# Autodesk Inventor assembly: Spool Holder V2.1
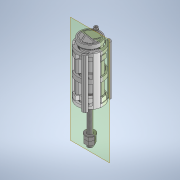
[picture p0: Inventor's stored thumbnail of the model, 180x180]
Saved by Autodesk Inventor 2020.3 (Build 243373010, 373A)
## iProperties
Created: 2021-07-05
Part Number: Spool Holder V2.1
Document SubType Name: Assembly
Designer: Parker
Author: Parker
## Documents named in this file (57)
- D:\Designs\MK3PRO P1\ACCESSORIES\Spool Holder V2\Spool Holder V2.1.iam
- D:\Designs\MK3PRO P1\ACCESSORIES\Spool Holder V2\M8 All Thread.ipt
- D:\Designs\MK3PRO P1\ACCESSORIES\Spool Holder V2\M8 Nut 6.ipt
- D:\Designs\MK3PRO P1\ACCESSORIES\Spool Holder V2\608RS Bearing.ipt
- D:\Designs\MK3PRO P1\ACCESSORIES\Spool Holder V2\M8 Washer.ipt
- D:\Designs\MK3PRO P1\ACCESSORIES\Spool Holder V2\M8 Nut 1.ipt
- D:\Designs\MK3PRO P1\ACCESSORIES\Spool Holder V2\M8 Washer 2.ipt
- D:\Designs\MK3PRO P1\ACCESSORIES\Spool Holder V2\M8 Nut 2.ipt
- D:\Designs\MK3PRO P1\ACCESSORIES\Spool Holder V2\M8 Nut 3.ipt
- D:\Designs\MK3PRO P1\ACCESSORIES\Spool Holder V2\M8 Washer 3.ipt
- D:\Designs\MK3PRO P1\ACCESSORIES\Spool Holder V2\608RS Bearing 2.ipt
- D:\Designs\MK3PRO P1\ACCESSORIES\Spool Holder V2\M8 Washer 4.ipt
- D:\Designs\MK3PRO P1\ACCESSORIES\Spool Holder V2\M8 Nut 4.ipt
- D:\Designs\MK3PRO P1\ACCESSORIES\Spool Holder V2\M8 Nut 5.ipt
- D:\Designs\MK3PRO P1\ACCESSORIES\Spool Holder V2\Pulley Body.ipt
- D:\Designs\MK3PRO P1\ACCESSORIES\Spool Holder V2\Moving Pin.ipt
- D:\Designs\MK3PRO P1\ACCESSORIES\Spool Holder V2\Stationary.ipt
- D:\Designs\MK3PRO P1\ACCESSORIES\Spool Holder V2\Solid17.ipt
- D:\Designs\MK3PRO P1\ACCESSORIES\Spool Holder V2\Solid18.ipt
- D:\Designs\MK3PRO P1\ACCESSORIES\Spool Holder V2\Rear Stator.ipt
- D:\Designs\MK3PRO P1\ACCESSORIES\Spool Holder V2\Rear Adjustor.ipt
- D:\Designs\MK3PRO P1\ACCESSORIES\Spool Holder V2\Bar3.ipt
- D:\Designs\MK3PRO P1\ACCESSORIES\Spool Holder V2\Bar2.ipt
- D:\Designs\MK3PRO P1\ACCESSORIES\Spool Holder V2\Bar1.ipt
- D:\Designs\MK3PRO P1\ACCESSORIES\Spool Holder V2\Solid41.ipt
- D:\Designs\MK3PRO P1\ACCESSORIES\Spool Holder V2\Solid40.ipt
- D:\Designs\MK3PRO P1\ACCESSORIES\Spool Holder V2\Solid38.ipt
- D:\Designs\MK3PRO P1\ACCESSORIES\Spool Holder V2\Solid39.ipt
- D:\Designs\MK3PRO P1\ACCESSORIES\Spool Holder V2\Solid29.ipt
- D:\Designs\MK3PRO P1\ACCESSORIES\Spool Holder V2\Solid31.ipt
- D:\Designs\MK3PRO P1\ACCESSORIES\Spool Holder V2\Solid30.ipt
- D:\Designs\MK3PRO P1\ACCESSORIES\Spool Holder V2\Solid32.ipt
- D:\Designs\MK3PRO P1\ACCESSORIES\Spool Holder V2\Solid33.ipt
- D:\Designs\MK3PRO P1\ACCESSORIES\Spool Holder V2\Solid37.ipt
- D:\Designs\MK3PRO P1\ACCESSORIES\Spool Holder V2\Solid36.ipt
- D:\Designs\MK3PRO P1\ACCESSORIES\Spool Holder V2\Solid34.ipt
- D:\Designs\MK3PRO P1\ACCESSORIES\Spool Holder V2\Solid35.ipt
- D:\Designs\MK3PRO P1\ACCESSORIES\Spool Holder V2\Solid25.ipt
- D:\Designs\MK3PRO P1\ACCESSORIES\Spool Holder V2\Solid42.ipt
- D:\Designs\MK3PRO P1\ACCESSORIES\Spool Holder V2\Solid28.ipt
- D:\Designs\MK3PRO P1\ACCESSORIES\Spool Holder V2\Solid26.ipt
- D:\Designs\MK3PRO P1\ACCESSORIES\Spool Holder V2\Solid27.ipt
- D:\Designs\MK3PRO P1\ACCESSORIES\Spool Holder V2\Solid43.ipt
- D:\Designs\MK3PRO P1\ACCESSORIES\Spool Holder V2\Solid24.ipt
- D:\Designs\MK3PRO P1\ACCESSORIES\Spool Holder V2\Front Cap.ipt
- D:\Designs\MK3PRO P1\ACCESSORIES\Spool Holder V2\Front Ratchet.ipt
- D:\Designs\MK3PRO P1\ACCESSORIES\Spool Holder V2\Lock Bar 6.ipt
- D:\Designs\MK3PRO P1\ACCESSORIES\Spool Holder V2\Lock Bar 4.ipt
- D:\Designs\MK3PRO P1\ACCESSORIES\Spool Holder V2\Lock Bar 1.ipt
- D:\Designs\MK3PRO P1\ACCESSORIES\Spool Holder V2\Lock Bar 2.ipt
- D:\Designs\MK3PRO P1\ACCESSORIES\Spool Holder V2\Lock Bar 5.ipt
- D:\Designs\MK3PRO P1\ACCESSORIES\Spool Holder V2\Lock Bar 3.ipt
- C:\Users\Parker\Documents\Inventor\Content Center Files\R2020\en-US\ANSI B18.22 M\ANSI B18.22M - 3 N.ipt
- C:\Users\Parker\Documents\Inventor\Content Center Files\R2020\en-US\ANSI B18.3.1M(6)\ANSI B18.3.1M - M3x0.5 x 10(1).ipt
- D:\Designs\MK3PRO P1\ACCESSORIES\Spool Holder V2\Solid53.ipt
- D:\Designs\MK3PRO P1\ACCESSORIES\Spool Holder V2\Solid55.ipt
- D:\Designs\MK3PRO P1\ACCESSORIES\Spool Holder V2\Solid54.ipt
## Components (68 placed, 56 different names)
1. M8 All Thread:1 — Mate:1, Mate:2, Mate:17, Mate:19, Mate:23, Mate:29, Mate:31, Mate:63
2. M8 Nut 6:1
3. 608RS Bearing:1 — Flush:10, Mate:20
4. M8 Washer:1
5. M8 Nut 1:1
6. M8 Washer 2:1
7. M8 Nut 2:1
8. M8 Nut 3:1
9. M8 Washer 3:1
10. 608RS Bearing 2:1 — Flush:2, Mate:32
11. M8 Washer 4:1
12. M8 Nut 4:1
13. M8 Nut 5:1 — Mate:60, Mate:61
14. Moving Pin:1 — Tangent:1, Tangent:2, Mate:5, Mate:6, Mate:8, Flush:3, Mate:10, Mate:52, Mate:54, Mate:57, Mate:58, Mate:81, Mate:83, Mate:89, Mate:90
15. Stationary:1 — Tangent:2, Flush:2, Mate:2, Mate:8, Mate:9, Tangent:3, Tangent:6, Mate:10, Flush:11, Angle:1, Angle:2, Angle:3, Mate:78, Mate:80, Mate:82, Mate:95
16. Solid17:1 — Tangent:3, Tangent:4, Flush:5, Mate:44, Mate:46, Mate:48, Mate:50, Mate:77, Mate:85, Mate:91, Mate:92
17. Solid18:1 — Tangent:5, Tangent:6, Flush:4, Mate:37, Mate:41, Mate:79, Mate:87, Mate:93, Mate:94
18. Rear Stator:1 — Mate:19, Flush:10, Flush:11, Mate:21, Mate:84, Mate:86, Mate:88
19. Rear Adjustor:1 — Mate:17, Flush:9, Mate:18
20. Bar3:1 — Mate:11, Mate:12, Flush:6, Flush:9, Mate:18
21. Bar2:1 — Mate:13, Mate:14, Flush:7, Mate:42
22. Bar1:1 — Mate:15, Mate:16, Flush:8
23. Pulley Body:1 — Mate:1, Tangent:1, Mate:5, Mate:6, Mate:9, Flush:3, Tangent:4, Tangent:5, Flush:4, Flush:5, Mate:11, Mate:12, Flush:6, Mate:13, Mate:14, Flush:7, Mate:15, Mate:16, Flush:8
24. Solid41:1 — Mate:45, Mate:46
25. Solid40:1 — Mate:43, Mate:44, Mate:45, Mate:71
26. Solid38:1 — Mate:47, Mate:48, Mate:49, Mate:69
27. Solid39:1 — Mate:49, Mate:50
28. Solid29:1 — Mate:34, Flush:12, Flush:13, Mate:38, Mate:42, Mate:43, Mate:47, Mate:51, Mate:55
29. Solid31:1 — Mate:53, Mate:54
30. Solid30:1 — Mate:51, Mate:52, Mate:53, Mate:75
31. Solid32:1 — Mate:55, Mate:56, Mate:58, Mate:73
32. Solid33:1 — Mate:56, Mate:57
33. Solid37:1 — Mate:39, Mate:40, Mate:41
34. Solid36:1 — Mate:38, Mate:39, Mate:40, Mate:65
35. Solid34:1 — Flush:13, Mate:35, Mate:36, Mate:67
36. Solid35:1 — Mate:35, Mate:36, Mate:37
37. Solid25:1 — Mate:32, Mate:33
38. Solid42:1 — Mate:30, Mate:31, Mate:33
39. Solid28:1 — Mate:28, Mate:29, Mate:30
40. Solid26:1 — Mate:26, Mate:27, Mate:28, Mate:34, Flush:12
41. Solid27:1 — Mate:24, Mate:25, Mate:26
42. Solid43:1 — Mate:22, Mate:23, Mate:24, Mate:25, Mate:27
43. Solid24:1 — Mate:20, Mate:21, Mate:22
44. Front Cap:1 — Mate:60, Mate:61, Mate:62, Mate:63, Mate:64, Insert:1
45. Front Ratchet:1 — Mate:62, Mate:64
46. Lock Bar 6:1 — Mate:71, Angle:3, Flush:14, Insert:8, Mate:91
47. Lock Bar 4:1 — Mate:69, Flush:14, Insert:4, Mate:92
48. Lock Bar 1:1 — Mate:67, Flush:15, Insert:5, Mate:94
49. Lock Bar 2:1 — Mate:65, Angle:2, Flush:15, Insert:7, Mate:93
50. Lock Bar 5:1 — Mate:75, Angle:1, Flush:16, Insert:6, Mate:89
51. Lock Bar 3:1 — Mate:73, Flush:16, Insert:3, Mate:90
52. Plain Washer (Metric) 3 N:1 — Insert:1, Insert:2
53. Forged Socket Head Cap Screw - Metric M3x0.5 x 10:1 — Insert:2
54. Plain Washer (Metric) 3 N:2 — Insert:3
55. Plain Washer (Metric) 3 N:3 — Insert:4
56. Plain Washer (Metric) 3 N:4 — Insert:5
57. Plain Washer (Metric) 3 N:5 — Insert:6
58. Plain Washer (Metric) 3 N:6 — Insert:7
59. Plain Washer (Metric) 3 N:7 — Insert:8
60. Plain Washer (Metric) 3 N:8 — Mate:77, Mate:78
61. Plain Washer (Metric) 3 N:9 — Mate:79, Mate:80
62. Plain Washer (Metric) 3 N:10 — Mate:81, Mate:82
63. Plain Washer (Metric) 3 N:11 — Mate:83, Mate:84
64. Plain Washer (Metric) 3 N:12 — Mate:85, Mate:86
65. Plain Washer (Metric) 3 N:13 — Mate:87, Mate:88
66. Solid53:1
67. Solid55:1
68. Solid54:1 — Mate:95
## Relationships (117: Mate 85, Flush 15, Insert 8, Tangent 6, Angle 3)
- Mate:1: M8 All Thread:1 ↔ Pulley Body:1
- Tangent:1: Moving Pin:1 ↔ Pulley Body:1
- Tangent:2: Moving Pin:1 ↔ Stationary:1
- Flush:2: 608RS Bearing 2:1 ↔ Stationary:1
- Mate:2: M8 All Thread:1 ↔ Stationary:1
- Mate:5: Moving Pin:1 ↔ Pulley Body:1
- Mate:6: Moving Pin:1 ↔ Pulley Body:1
- Mate:8: Moving Pin:1 ↔ Stationary:1
- Mate:9 (2 mm): Stationary:1 ↔ Pulley Body:1
- Flush:3: Moving Pin:1 ↔ Pulley Body:1
- Tangent:3: Stationary:1 ↔ Solid17:1
- Tangent:4: Solid17:1 ↔ Pulley Body:1
- Tangent:5: Solid18:1 ↔ Pulley Body:1
- Tangent:6: Stationary:1 ↔ Solid18:1
- Flush:4: Solid18:1 ↔ Pulley Body:1
- Flush:5: Solid17:1 ↔ Pulley Body:1
- Mate:10: Moving Pin:1 ↔ Stationary:1
- Mate:11: Bar3:1 ↔ Pulley Body:1
- Mate:12: Bar3:1 ↔ Pulley Body:1
- Flush:6: Bar3:1 ↔ Pulley Body:1
- Mate:13: Bar2:1 ↔ Pulley Body:1
- Mate:14: Bar2:1 ↔ Pulley Body:1
- Flush:7: Bar2:1 ↔ Pulley Body:1
- Mate:15: Bar1:1 ↔ Pulley Body:1
- Mate:16: Bar1:1 ↔ Pulley Body:1
- Flush:8: Bar1:1 ↔ Pulley Body:1
- Mate:17: M8 All Thread:1 ↔ Rear Adjustor:1
- Flush:9: Rear Adjustor:1 ↔ Bar3:1
- Mate:18: Rear Adjustor:1 ↔ Bar3:1
- Mate:19: M8 All Thread:1 ↔ Rear Stator:1
- Flush:10: 608RS Bearing:1 ↔ Rear Stator:1
- Flush:11: Stationary:1 ↔ Rear Stator:1
- Mate:20: 608RS Bearing:1 ↔ Solid24:1
- Mate:21: Rear Stator:1 ↔ Solid24:1
- Mate:22: Solid43:1 ↔ Solid24:1
- Mate:23: M8 All Thread:1 ↔ Solid43:1
- Mate:24: Solid27:1 ↔ Solid43:1
- Mate:25: Solid27:1 ↔ Solid43:1
- Mate:26: Solid26:1 ↔ Solid27:1
- Mate:27: Solid26:1 ↔ Solid43:1
- Mate:28: Solid28:1 ↔ Solid26:1
- Mate:29: M8 All Thread:1 ↔ Solid28:1
- Mate:30: Solid42:1 ↔ Solid28:1
- Mate:31: M8 All Thread:1 ↔ Solid42:1
- Mate:32: 608RS Bearing 2:1 ↔ Solid25:1
- Mate:33: Solid25:1 ↔ Solid42:1
- Mate:34: Solid29:1 ↔ Solid26:1
- Flush:12: Solid29:1 ↔ Solid26:1
- Flush:13 (-1 mm): Solid29:1 ↔ Solid34:1
- Mate:35: Solid34:1 ↔ Solid35:1
- Mate:36: Solid34:1 ↔ Solid35:1
- Mate:37: Solid18:1 ↔ Solid35:1
- Mate:38 (1 mm): Solid29:1 ↔ Solid36:1
- Mate:39: Solid37:1 ↔ Solid36:1
- Mate:40: Solid37:1 ↔ Solid36:1
- Mate:41: Solid18:1 ↔ Solid37:1
- Mate:42: Bar2:1 ↔ Solid29:1
- Mate:43 (1 mm): Solid40:1 ↔ Solid29:1
- Mate:44: Solid17:1 ↔ Solid40:1
- Mate:45: Solid41:1 ↔ Solid40:1
- Mate:46: Solid17:1 ↔ Solid41:1
- Mate:47 (1 mm): Solid38:1 ↔ Solid29:1
- Mate:48: Solid17:1 ↔ Solid38:1
- Mate:49: Solid38:1 ↔ Solid39:1
- Mate:50: Solid17:1 ↔ Solid39:1
- Mate:51: Solid29:1 ↔ Solid30:1
- Mate:52: Moving Pin:1 ↔ Solid30:1
- Mate:53: Solid31:1 ↔ Solid30:1
- Mate:54: Moving Pin:1 ↔ Solid31:1
- Mate:55 (1 mm): Solid29:1 ↔ Solid32:1
- Mate:56: Solid32:1 ↔ Solid33:1
- Mate:57: Moving Pin:1 ↔ Solid33:1
- Mate:58: Moving Pin:1 ↔ Solid32:1
- Mate:60: M8 Nut 5:1 ↔ Front Cap:1
- Mate:61: M8 Nut 5:1 ↔ Front Cap:1
- Mate:62 (0.5 mm): Front Cap:1 ↔ Front Ratchet:1
- Mate:63 (1 mm): M8 All Thread:1 ↔ Front Cap:1
- Mate:64: Front Cap:1 ↔ Front Ratchet:1
- Insert:1: Front Cap:1 ↔ Plain Washer (Metric) 3 N:1
- Insert:2: Plain Washer (Metric) 3 N:1 ↔ Forged Socket Head Cap Screw - Metric M3x0.5 x 10:1
- Mate:65: Solid36:1 ↔ Lock Bar 2:1
- Mate:67: Solid34:1 ↔ Lock Bar 1:1
- Mate:69: Solid38:1 ↔ Lock Bar 4:1
- Mate:71: Solid40:1 ↔ Lock Bar 6:1
- Mate:73: Solid32:1 ↔ Lock Bar 3:1
- Mate:75: Solid30:1 ↔ Lock Bar 5:1
- Angle:1 (0 deg): Stationary:1 ↔ Lock Bar 5:1
- Angle:2 (0 deg): Stationary:1 ↔ Lock Bar 2:1
- Angle:3 (0 deg): Stationary:1 ↔ Lock Bar 6:1
- Flush:14: Lock Bar 6:1 ↔ Lock Bar 4:1
- Flush:15: Lock Bar 1:1 ↔ Lock Bar 2:1
- Flush:16: Lock Bar 5:1 ↔ Lock Bar 3:1
- Insert:3: Lock Bar 3:1 ↔ Plain Washer (Metric) 3 N:2
- Insert:4: Lock Bar 4:1 ↔ Plain Washer (Metric) 3 N:3
- Insert:5: Lock Bar 1:1 ↔ Plain Washer (Metric) 3 N:4
- Insert:6: Lock Bar 5:1 ↔ Plain Washer (Metric) 3 N:5
- Insert:7: Lock Bar 2:1 ↔ Plain Washer (Metric) 3 N:6
- Insert:8: Lock Bar 6:1 ↔ Plain Washer (Metric) 3 N:7
- Mate:77: Solid17:1 ↔ Plain Washer (Metric) 3 N:8
- Mate:78: Stationary:1 ↔ Plain Washer (Metric) 3 N:8
- Mate:79: Solid18:1 ↔ Plain Washer (Metric) 3 N:9
- Mate:80: Stationary:1 ↔ Plain Washer (Metric) 3 N:9
- Mate:81: Moving Pin:1 ↔ Plain Washer (Metric) 3 N:10
- Mate:82: Stationary:1 ↔ Plain Washer (Metric) 3 N:10
- Mate:83: Moving Pin:1 ↔ Plain Washer (Metric) 3 N:11
- Mate:84: Rear Stator:1 ↔ Plain Washer (Metric) 3 N:11
- Mate:85: Solid17:1 ↔ Plain Washer (Metric) 3 N:12
- Mate:86: Rear Stator:1 ↔ Plain Washer (Metric) 3 N:12
- Mate:87: Solid18:1 ↔ Plain Washer (Metric) 3 N:13
- Mate:88: Rear Stator:1 ↔ Plain Washer (Metric) 3 N:13
- Mate:89: Moving Pin:1 ↔ Lock Bar 5:1
- Mate:90: Moving Pin:1 ↔ Lock Bar 3:1
- Mate:91: Solid17:1 ↔ Lock Bar 6:1
- Mate:92: Solid17:1 ↔ Lock Bar 4:1
- Mate:93: Solid18:1 ↔ Lock Bar 2:1
- Mate:94: Solid18:1 ↔ Lock Bar 1:1
- Mate:95: Stationary:1 ↔ Solid54:1
